# Autodesk Inventor assembly: ASY GBK 0070 bottom 70
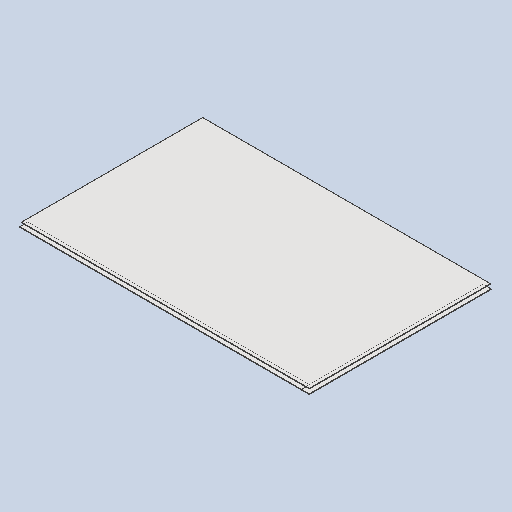
[picture p0: Inventor's stored thumbnail of the model, 512x512]
Saved by Autodesk Inventor 2026.2 (Build 302298000, 298)
## iProperties
Created: 2026-07-16
Part Number: ASY GBK 0070 bottom 70
Document SubType Name: Assembly
Designer: user
Stock Number: 0070
Author: user
## Documents named in this file (4)
- C:\Users\admin\Documents\Inventor\GBK-Gubkinskiy\ASY GBK bottom 0024.iam
- C:\Users\admin\Documents\Inventor\GBK-Gubkinskiy\Пол\GBK bottom 0231.ipt
- C:\Users\admin\Documents\Inventor\GBK-Gubkinskiy\Пол\GBK bottom 0131.ipt
- C:\Users\admin\Documents\Inventor\GBK-Gubkinskiy\Пол\GBK bottom 0134.ipt
## Components (3 placed, 3 different names)
1. GBK bottom 0231:1
2. GBK bottom 0131:1
3. GBK bottom 0134:1
## Relationships (4: Mate 3, WeldJoint 1)
- [WeldJoint]: GBK bottom 0131:1 ↔ GBK bottom 0134:1
- [Mate]: GBK bottom 0231:1 ↔ GBK bottom 0134:1
- [Mate] (-30 mm): GBK bottom 0231:1 ↔ GBK bottom 0134:1
- [Mate] (-30 mm): GBK bottom 0231:1 ↔ GBK bottom 0131:1
